# Autodesk Inventor assembly: Hopper Sheet Metal assy
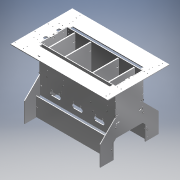
[picture p0: Inventor's stored thumbnail of the model, 180x180]
Saved by Autodesk Inventor 2018 (Build 220112000, 112)
## iProperties
Created: 2017-09-21
Part Number: Hopper Sheet Metal assy
Document SubType Name: Assembly
Designer: Gabriel Smolnycki
Author: Gabriel Smolnycki
## Documents named in this file (12)
- E:\planb\mechanics\V1INV\Subassemblies\Hopper Sheet Metal assy.iam
- E:\planb\mechanics\V1INV\Hopper\Hopper Bottom Brace.ipt
- E:\planb\mechanics\V1INV\Hopper\Hopper Wall.ipt
- E:\planb\mechanics\V1INV\Hopper\Hopper Side.ipt
- E:\planb\mechanics\V1INV\Hopper\Hopper Feed Wall.ipt
- E:\planb\mechanics\V1INV\Hopper\Hopper Outer Wall.ipt
- E:\planb\mechanics\V1INV\Hopper\Hopper Outer Wall with Megatronics mount.ipt
- E:\planb\mechanics\V1INV\Hopper\Hopper Leg Brace.ipt
- E:\planb\mechanics\V1INV\Hopper\Hopper Top.ipt
- E:\planb\mechanics\V1INV\Hardware\M3 SS Nut.ipt
- E:\planb\mechanics\V1INV\Hardware\M3 SS Washer.ipt
- E:\planb\mechanics\V1INV\Hardware\M3x16 SS SHCS.ipt
## Components (150 placed, 11 different names)
1. Hopper Bottom Brace:1 — Mate:1, Mate:2, Mate:3, Mate:4, Mate:5, Mate:6, Mate:40, Mate:43, Mate:52, Mate:54, Insert:28, Insert:33
2. Hopper Wall:1 — Mate:1, Mate:2, Mate:3, Mate:7, Mate:8, Mate:9
3. Hopper Wall:2 — Mate:4, Mate:5, Mate:6, Mate:16, Mate:17, Mate:18, Mate:38, Mate:39, Mate:41, Mate:42, Mate:53, Mate:55
4. Hopper Side:1 — Mate:7, Mate:8, Mate:9, Mate:10, Mate:11, Mate:12, Mate:13, Mate:14, Mate:15, Mate:19, Mate:20, Mate:21, Mate:22, Mate:23, Mate:24, Insert:1, Insert:2, Insert:3, Insert:4, Insert:5, Mate:46, Mate:50, Insert:8, Insert:9, Insert:21, Insert:22, Insert:23, Insert:24, Insert:25, Insert:26, Insert:27
5. Hopper Feed Wall:1 — Mate:10, Mate:11, Mate:12, Mate:34, Mate:35, Mate:36, Mate:37, Insert:29, Insert:31
6. Hopper Feed Wall:2 — Mate:13, Mate:14, Mate:15
7. Hopper Side:2 — Mate:16, Mate:17, Mate:18
8. Hopper Outer Wall:1 — Mate:22, Mate:23, Mate:24, Mate:25, Mate:26, Mate:27, Mate:28, Mate:29, Mate:30, Mate:44, Mate:45, Mate:48, Mate:49, Insert:6, Insert:7, Insert:19, Insert:20, Mate:56, Mate:57
9. Hopper Outer Wall with Megatronics mount:1 — Mate:19, Mate:20, Mate:21, Mate:31, Mate:32, Mate:33
10. Hopper Leg Brace:1 — Mate:25, Mate:26, Mate:27, Mate:47, Mate:51
11. Hopper Leg Brace:2 — Mate:28, Mate:29, Mate:30
12. Hopper Top:1 — Mate:31, Mate:32, Mate:33, Insert:67, Insert:68
13. M3 SS Nut:1 — Mate:40, Mate:43, Insert:5
14. M3 SS Nut:2 — Mate:39, Mate:42, Insert:4
15. M3 SS Nut:3 — Mate:38, Mate:41, Insert:3
16. M3 SS Nut:4 — Mate:36, Mate:37, Insert:2
17. M3 SS Nut:5 — Mate:34, Mate:35, Insert:1
18. M3 SS Nut:6 — Mate:45, Mate:49, Insert:9
19. M3 SS Nut:7 — Mate:47, Mate:51, Insert:6
20. M3 SS Nut:8 — Mate:46, Mate:50, Insert:7
21. M3 SS Nut:9 — Mate:44, Mate:48, Insert:8
22. M3 SS Nut:10 — Mate:52, Mate:54, Insert:29
23. M3 SS Nut:11 — Mate:53, Mate:55, Insert:28
24. M3 SS Washer:1 — Insert:18, Insert:19
25. M3 SS Washer:2 — Insert:17, Insert:20
26. M3 SS Washer:3 — Insert:16, Insert:21
27. M3 SS Washer:4 — Insert:15, Insert:22
28. M3 SS Washer:5 — Insert:14, Insert:23
29. M3 SS Washer:6 — Insert:13, Insert:24
30. M3 SS Washer:7 — Insert:12, Insert:25
31. M3 SS Washer:8 — Insert:11, Insert:26
32. M3 SS Washer:9 — Insert:10, Insert:27
33. M3 SS Washer:10 — Insert:30, Insert:31
34. M3 SS Washer:11 — Insert:32, Insert:33
35. M3x16 SS SHCS:1 — Insert:18
36. M3x16 SS SHCS:2 — Insert:17
37. M3x16 SS SHCS:3 — Insert:16
38. M3x16 SS SHCS:4 — Insert:15
39. M3x16 SS SHCS:5 — Insert:14
40. M3x16 SS SHCS:6 — Insert:13
41. M3x16 SS SHCS:7 — Insert:12
42. M3x16 SS SHCS:8 — Insert:11
43. M3x16 SS SHCS:9 — Insert:10
44. M3x16 SS SHCS:10 — Insert:30
45. M3x16 SS SHCS:11 — Insert:32
46. M3 SS Nut:12
47. M3 SS Nut:13
48. M3 SS Nut:14
49. M3 SS Nut:15
50. M3 SS Nut:16
51. M3 SS Nut:17
52. M3 SS Nut:18
53. M3 SS Nut:19
54. M3 SS Nut:20
55. M3 SS Nut:21
56. M3 SS Nut:22
57. M3 SS Washer:12 — Insert:34
58. M3 SS Washer:13 — Insert:35
59. M3 SS Washer:14 — Insert:36
60. M3 SS Washer:15 — Insert:37
61. M3 SS Washer:16 — Insert:38
62. M3 SS Washer:17 — Insert:39
63. M3 SS Washer:18 — Insert:40
64. M3 SS Washer:19 — Insert:41
65. M3 SS Washer:20 — Insert:42
66. M3 SS Washer:21 — Insert:43
67. M3 SS Washer:22 — Insert:44
68. M3x16 SS SHCS:12 — Insert:34
69. M3x16 SS SHCS:13 — Insert:35
70. M3x16 SS SHCS:14 — Insert:36
71. M3x16 SS SHCS:15 — Insert:37
72. M3x16 SS SHCS:16 — Insert:38
73. M3x16 SS SHCS:17 — Insert:39
74. M3x16 SS SHCS:18 — Insert:40
75. M3x16 SS SHCS:19 — Insert:41
76. M3x16 SS SHCS:20 — Insert:42
77. M3x16 SS SHCS:21 — Insert:43
78. M3x16 SS SHCS:22 — Insert:44
79. M3 SS Nut:23
80. M3 SS Nut:24
81. M3 SS Nut:25
82. M3 SS Nut:26
83. M3 SS Nut:27
84. M3 SS Nut:28
85. M3 SS Nut:29
86. M3 SS Nut:30
87. M3 SS Nut:31
88. M3 SS Nut:32
89. M3 SS Nut:33
90. M3 SS Washer:23 — Insert:45
91. M3 SS Washer:24 — Insert:46
92. M3 SS Washer:25 — Insert:47
93. M3 SS Washer:26 — Insert:48
94. M3 SS Washer:27 — Insert:49
95. M3 SS Washer:28 — Insert:50
96. M3 SS Washer:29 — Insert:51
97. M3 SS Washer:30 — Insert:52
98. M3 SS Washer:31 — Insert:53
99. M3 SS Washer:32 — Insert:54
100. M3 SS Washer:33 — Insert:55
101. M3x16 SS SHCS:23 — Insert:45
102. M3x16 SS SHCS:24 — Insert:46
103. M3x16 SS SHCS:25 — Insert:47
104. M3x16 SS SHCS:26 — Insert:48
105. M3x16 SS SHCS:27 — Insert:49
106. M3x16 SS SHCS:28 — Insert:50
107. M3x16 SS SHCS:29 — Insert:51
108. M3x16 SS SHCS:30 — Insert:52
109. M3x16 SS SHCS:31 — Insert:53
110. M3x16 SS SHCS:32 — Insert:54
111. M3x16 SS SHCS:33 — Insert:55
112. M3 SS Nut:34
113. M3 SS Nut:35
114. M3 SS Nut:36
115. M3 SS Nut:37
116. M3 SS Nut:38
117. M3 SS Nut:39
118. M3 SS Nut:40
119. M3 SS Nut:41
120. M3 SS Nut:42
121. M3 SS Nut:43
122. M3 SS Nut:44
123. M3 SS Washer:34 — Insert:56
124. M3 SS Washer:35 — Insert:57
125. M3 SS Washer:36 — Insert:58
126. M3 SS Washer:37 — Insert:59
127. M3 SS Washer:38 — Insert:60
128. M3 SS Washer:39 — Insert:61
129. M3 SS Washer:40 — Insert:62
130. M3 SS Washer:41 — Insert:63
131. M3 SS Washer:42 — Insert:64
132. M3 SS Washer:43 — Insert:65
133. M3 SS Washer:44 — Insert:66
134. M3x16 SS SHCS:34 — Insert:56
135. M3x16 SS SHCS:35 — Insert:57
136. M3x16 SS SHCS:36 — Insert:58
137. M3x16 SS SHCS:37 — Insert:59
138. M3x16 SS SHCS:38 — Insert:60
139. M3x16 SS SHCS:39 — Insert:61
140. M3x16 SS SHCS:40 — Insert:62
141. M3x16 SS SHCS:41 — Insert:63
142. M3x16 SS SHCS:42 — Insert:64
143. M3x16 SS SHCS:43 — Insert:65
144. M3x16 SS SHCS:44 — Insert:66
145. M3 SS Nut:45 — Mate:56, Mate:57, Insert:67
146. M3 SS Washer:45 — Insert:68, Insert:69
147. M3x16 SS SHCS:45 — Insert:69
148. M3 SS Nut:46
149. M3 SS Washer:46 — Insert:70
150. M3x16 SS SHCS:46 — Insert:70
## Relationships (127: Insert 70, Mate 57)
- Mate:1 (0.3969 mm): Hopper Bottom Brace:1 ↔ Hopper Wall:1
- Mate:2 (1 mm): Hopper Bottom Brace:1 ↔ Hopper Wall:1
- Mate:3: Hopper Bottom Brace:1 ↔ Hopper Wall:1
- Mate:4 (1 mm): Hopper Bottom Brace:1 ↔ Hopper Wall:2
- Mate:5 (0.3969 mm): Hopper Bottom Brace:1 ↔ Hopper Wall:2
- Mate:6: Hopper Bottom Brace:1 ↔ Hopper Wall:2
- Mate:7 (0.1984 mm): Hopper Wall:1 ↔ Hopper Side:1
- Mate:8 (0.5 mm): Hopper Wall:1 ↔ Hopper Side:1
- Mate:9: Hopper Wall:1 ↔ Hopper Side:1
- Mate:10 (0.1984 mm): Hopper Side:1 ↔ Hopper Feed Wall:1
- Mate:11 (0.5 mm): Hopper Side:1 ↔ Hopper Feed Wall:1
- Mate:12: Hopper Side:1 ↔ Hopper Feed Wall:1
- Mate:13 (0.1984 mm): Hopper Side:1 ↔ Hopper Feed Wall:2
- Mate:14 (0.5 mm): Hopper Side:1 ↔ Hopper Feed Wall:2
- Mate:15: Hopper Side:1 ↔ Hopper Feed Wall:2
- Mate:16 (0.1984 mm): Hopper Wall:2 ↔ Hopper Side:2
- Mate:17 (0.5 mm): Hopper Wall:2 ↔ Hopper Side:2
- Mate:18: Hopper Wall:2 ↔ Hopper Side:2
- Mate:19 (0.5 mm): Hopper Side:1 ↔ Hopper Outer Wall with Megatronics mount:1
- Mate:20: Hopper Side:1 ↔ Hopper Outer Wall with Megatronics mount:1
- Mate:21: Hopper Side:1 ↔ Hopper Outer Wall with Megatronics mount:1
- Mate:22 (1 mm): Hopper Side:1 ↔ Hopper Outer Wall:1
- Mate:23: Hopper Side:1 ↔ Hopper Outer Wall:1
- Mate:24: Hopper Side:1 ↔ Hopper Outer Wall:1
- Mate:25 (0.25 mm): Hopper Outer Wall:1 ↔ Hopper Leg Brace:1
- Mate:26 (0.1984 mm): Hopper Outer Wall:1 ↔ Hopper Leg Brace:1
- Mate:27: Hopper Outer Wall:1 ↔ Hopper Leg Brace:1
- Mate:28 (0.25 mm): Hopper Outer Wall:1 ↔ Hopper Leg Brace:2
- Mate:29 (0.1984 mm): Hopper Outer Wall:1 ↔ Hopper Leg Brace:2
- Mate:30: Hopper Outer Wall:1 ↔ Hopper Leg Brace:2
- Mate:31 (0.5 mm): Hopper Outer Wall with Megatronics mount:1 ↔ Hopper Top:1
- Mate:32 (0.3969 mm): Hopper Outer Wall with Megatronics mount:1 ↔ Hopper Top:1
- Mate:33: Hopper Outer Wall with Megatronics mount:1 ↔ Hopper Top:1
- Mate:34: Hopper Feed Wall:1 ↔ M3 SS Nut:5
- Mate:35: Hopper Feed Wall:1 ↔ M3 SS Nut:5
- Insert:1: Hopper Side:1 ↔ M3 SS Nut:5
- Mate:36: Hopper Feed Wall:1 ↔ M3 SS Nut:4
- Mate:37: Hopper Feed Wall:1 ↔ M3 SS Nut:4
- Insert:2: Hopper Side:1 ↔ M3 SS Nut:4
- Mate:38: Hopper Wall:2 ↔ M3 SS Nut:3
- Mate:39: Hopper Wall:2 ↔ M3 SS Nut:2
- Mate:40: Hopper Bottom Brace:1 ↔ M3 SS Nut:1
- Mate:41: Hopper Wall:2 ↔ M3 SS Nut:3
- Mate:42: Hopper Wall:2 ↔ M3 SS Nut:2
- Mate:43: Hopper Bottom Brace:1 ↔ M3 SS Nut:1
- Insert:3: Hopper Side:1 ↔ M3 SS Nut:3
- Insert:4: Hopper Side:1 ↔ M3 SS Nut:2
- Insert:5: Hopper Side:1 ↔ M3 SS Nut:1
- Mate:44: Hopper Outer Wall:1 ↔ M3 SS Nut:9
- Mate:45: Hopper Outer Wall:1 ↔ M3 SS Nut:6
- Mate:46: Hopper Side:1 ↔ M3 SS Nut:8
- Mate:47: Hopper Leg Brace:1 ↔ M3 SS Nut:7
- Mate:48: Hopper Outer Wall:1 ↔ M3 SS Nut:9
- Mate:49: Hopper Outer Wall:1 ↔ M3 SS Nut:6
- Mate:50: Hopper Side:1 ↔ M3 SS Nut:8
- Mate:51: Hopper Leg Brace:1 ↔ M3 SS Nut:7
- Insert:6: Hopper Outer Wall:1 ↔ M3 SS Nut:7
- Insert:7: Hopper Outer Wall:1 ↔ M3 SS Nut:8
- Insert:8: Hopper Side:1 ↔ M3 SS Nut:9
- Insert:9: Hopper Side:1 ↔ M3 SS Nut:6
- Insert:10: M3 SS Washer:9 ↔ M3x16 SS SHCS:9
- Insert:11: M3 SS Washer:8 ↔ M3x16 SS SHCS:8
- Insert:12: M3 SS Washer:7 ↔ M3x16 SS SHCS:7
- Insert:13: M3 SS Washer:6 ↔ M3x16 SS SHCS:6
- Insert:14: M3 SS Washer:5 ↔ M3x16 SS SHCS:5
- Insert:15: M3 SS Washer:4 ↔ M3x16 SS SHCS:4
- Insert:16: M3 SS Washer:3 ↔ M3x16 SS SHCS:3
- Insert:17: M3 SS Washer:2 ↔ M3x16 SS SHCS:2
- Insert:18: M3 SS Washer:1 ↔ M3x16 SS SHCS:1
- Insert:19: Hopper Outer Wall:1 ↔ M3 SS Washer:1
- Insert:20: Hopper Outer Wall:1 ↔ M3 SS Washer:2
- Insert:21: Hopper Side:1 ↔ M3 SS Washer:3
- Insert:22: Hopper Side:1 ↔ M3 SS Washer:4
- Insert:23: Hopper Side:1 ↔ M3 SS Washer:5
- Insert:24: Hopper Side:1 ↔ M3 SS Washer:6
- Insert:25: Hopper Side:1 ↔ M3 SS Washer:7
- Insert:26: Hopper Side:1 ↔ M3 SS Washer:8
- Insert:27: Hopper Side:1 ↔ M3 SS Washer:9
- Mate:52: Hopper Bottom Brace:1 ↔ M3 SS Nut:10
- Mate:53: Hopper Wall:2 ↔ M3 SS Nut:11
- Mate:54: Hopper Bottom Brace:1 ↔ M3 SS Nut:10
- Mate:55: Hopper Wall:2 ↔ M3 SS Nut:11
- Insert:28: Hopper Bottom Brace:1 ↔ M3 SS Nut:11
- Insert:29: Hopper Feed Wall:1 ↔ M3 SS Nut:10
- Insert:30: M3 SS Washer:10 ↔ M3x16 SS SHCS:10
- Insert:31: Hopper Feed Wall:1 ↔ M3 SS Washer:10
- Insert:32: M3 SS Washer:11 ↔ M3x16 SS SHCS:11
- Insert:33: Hopper Bottom Brace:1 ↔ M3 SS Washer:11
- Insert:34: M3 SS Washer:12 ↔ M3x16 SS SHCS:12
- Insert:35: M3 SS Washer:13 ↔ M3x16 SS SHCS:13
- Insert:36: M3 SS Washer:14 ↔ M3x16 SS SHCS:14
- Insert:37: M3 SS Washer:15 ↔ M3x16 SS SHCS:15
- Insert:38: M3 SS Washer:16 ↔ M3x16 SS SHCS:16
- Insert:39: M3 SS Washer:17 ↔ M3x16 SS SHCS:17
- Insert:40: M3 SS Washer:18 ↔ M3x16 SS SHCS:18
- Insert:41: M3 SS Washer:19 ↔ M3x16 SS SHCS:19
- Insert:42: M3 SS Washer:20 ↔ M3x16 SS SHCS:20
- Insert:43: M3 SS Washer:21 ↔ M3x16 SS SHCS:21
- Insert:44: M3 SS Washer:22 ↔ M3x16 SS SHCS:22
- Insert:45: M3 SS Washer:23 ↔ M3x16 SS SHCS:23
- Insert:46: M3 SS Washer:24 ↔ M3x16 SS SHCS:24
- Insert:47: M3 SS Washer:25 ↔ M3x16 SS SHCS:25
- Insert:48: M3 SS Washer:26 ↔ M3x16 SS SHCS:26
- Insert:49: M3 SS Washer:27 ↔ M3x16 SS SHCS:27
- Insert:50: M3 SS Washer:28 ↔ M3x16 SS SHCS:28
- Insert:51: M3 SS Washer:29 ↔ M3x16 SS SHCS:29
- Insert:52: M3 SS Washer:30 ↔ M3x16 SS SHCS:30
- Insert:53: M3 SS Washer:31 ↔ M3x16 SS SHCS:31
- Insert:54: M3 SS Washer:32 ↔ M3x16 SS SHCS:32
- Insert:55: M3 SS Washer:33 ↔ M3x16 SS SHCS:33
- Insert:56: M3 SS Washer:34 ↔ M3x16 SS SHCS:34
- Insert:57: M3 SS Washer:35 ↔ M3x16 SS SHCS:35
- Insert:58: M3 SS Washer:36 ↔ M3x16 SS SHCS:36
- Insert:59: M3 SS Washer:37 ↔ M3x16 SS SHCS:37
- Insert:60: M3 SS Washer:38 ↔ M3x16 SS SHCS:38
- Insert:61: M3 SS Washer:39 ↔ M3x16 SS SHCS:39
- Insert:62: M3 SS Washer:40 ↔ M3x16 SS SHCS:40
- Insert:63: M3 SS Washer:41 ↔ M3x16 SS SHCS:41
- Insert:64: M3 SS Washer:42 ↔ M3x16 SS SHCS:42
- Insert:65: M3 SS Washer:43 ↔ M3x16 SS SHCS:43
- Insert:66: M3 SS Washer:44 ↔ M3x16 SS SHCS:44
- Mate:56: Hopper Outer Wall:1 ↔ M3 SS Nut:45
- Mate:57: Hopper Outer Wall:1 ↔ M3 SS Nut:45
- Insert:67: Hopper Top:1 ↔ M3 SS Nut:45
- Insert:68: Hopper Top:1 ↔ M3 SS Washer:45
- Insert:69: M3 SS Washer:45 ↔ M3x16 SS SHCS:45
- Insert:70: M3 SS Washer:46 ↔ M3x16 SS SHCS:46
